# Autodesk Inventor assembly: Assembly1
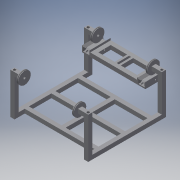
[picture p0: Inventor's stored thumbnail of the model, 180x180]
Saved by Autodesk Inventor 2016 (Build 200138000, 138)
## iProperties
Created: 2017-08-14
Part Number: Assembly1
Document SubType Name: Assembly
Designer: andre
Author: andre
## Documents named in this file (5)
- D:\Dropbox\AarhusUNI\Andet 2017\OrbitRaket\Assembly1.iam
- D:\Dropbox\AarhusUNI\Andet 2017\OrbitRaket\Raket_Arme.ipt
- D:\Dropbox\AarhusUNI\Andet 2017\OrbitRaket\Raket_Hjul.ipt
- D:\Dropbox\AarhusUNI\Andet 2017\OrbitRaket\Raket_Holder.ipt
- D:\Dropbox\AarhusUNI\Andet 2017\OrbitRaket\Raket_Lednings_Holder.ipt
## Components (10 placed, 4 different names)
1. Raket_Arme:1 — Rigid:1, Rotational:4
2. Raket_Holder:1 — Rigid:1, Rotational:1, Rotational:2, Rotational:3
3. Raket_Lednings_Holder:1
4. Raket_Arme:2 — Rotational:2, Rotational:5
5. Raket_Arme:3 — Rotational:3, Rotational:7
6. Raket_Arme:4 — Rotational:1, Rotational:6
7. Raket_Hjul:1 — Rotational:7
8. Raket_Hjul:2 — Rotational:6
9. Raket_Hjul:3 — Rotational:4
10. Raket_Hjul:4 — Rotational:5
## Relationships (8: RevoluteJoint 7, WeldJoint 1)
- Rigid:1 [WeldJoint]: Raket_Arme:1 ↔ Raket_Holder:1
- Rotational:1 [RevoluteJoint]: Raket_Holder:1 ↔ Raket_Arme:4
- Rotational:2 [RevoluteJoint]: Raket_Holder:1 ↔ Raket_Arme:2
- Rotational:3 [RevoluteJoint]: Raket_Holder:1 ↔ Raket_Arme:3
- Rotational:4 [RevoluteJoint]: Raket_Arme:1 ↔ Raket_Hjul:3
- Rotational:5 [RevoluteJoint]: Raket_Arme:2 ↔ Raket_Hjul:4
- Rotational:6 [RevoluteJoint]: Raket_Arme:4 ↔ Raket_Hjul:2
- Rotational:7 [RevoluteJoint]: Raket_Arme:3 ↔ Raket_Hjul:1
